# Autodesk Inventor assembly: Übertragung des Zahnriemens
Saved by Autodesk Inventor 2016 (Build 200138000, 138)
## iProperties
Created: 2015-08-24
Part Number: Übertragung des Zahnriemens
Document SubType Name: Assembly
Designer: 4ndreas
Mass: 547.527 g
Surface Area: 273.796 cm^2
Volume: 74.331 cm^3
Density: 7.36607 g/cm^3
ClientObjectVersion: 1
Author: 4ndreas
## Documents named in this file (4)
- C:\Users\4ndreas\Documents\Inventor\RobotARM v2\v4\Shoulder_stepper\Konstruktions-Assistent\Übertragung des Zahnriemens1.iam
- C:\Users\4ndreas\Documents\Inventor\RobotARM v2\v4\Shoulder_stepper\Konstruktions-Assistent\Zahnriemen1.ipt
- C:\Users\4ndreas\Documents\Inventor\RobotARM v2\v4\Shoulder_stepper\Konstruktions-Assistent\Flache Riemenscheibe21.ipt
- C:\Users\4ndreas\Documents\Inventor\RobotARM v2\v4\Shoulder_stepper\Konstruktions-Assistent\Flache Riemenscheibe11.ipt
## Components (3 placed, 3 different names)
1. Zahnriemen:1 — Fluchtend:1, Passend:1, Fluchtend:2, Passend:2
2. Flache Riemenscheibe2:1 — Fluchtend:1, Passend:1
3. Flache Riemenscheibe1:1 — Fluchtend:2, Passend:2
## Relationships (4: Flush 2, Mate 2)
- Fluchtend:1 [Flush] (1.3 mm): Zahnriemen:1 ↔ Flache Riemenscheibe2:1
- Passend:1 [Mate]: Zahnriemen:1 ↔ Flache Riemenscheibe2:1
- Fluchtend:2 [Flush] (1.3 mm): Zahnriemen:1 ↔ Flache Riemenscheibe1:1
- Passend:2 [Mate]: Zahnriemen:1 ↔ Flache Riemenscheibe1:1
